# Autodesk Inventor assembly: Assembly2finalfinal
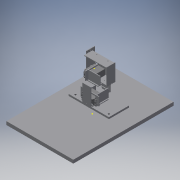
[picture p0: Inventor's stored thumbnail of the model, 180x180]
Saved by Autodesk Inventor 2019 (Build 230136000, 136)
## iProperties
Created: 2020-02-29
Part Number: Assembly2finalfinal
Document SubType Name: Assembly
Designer: Hp
Author: Hp
## Documents named in this file (14)
- C:\Users\Hp\Desktop\siri revant\final3ddiagrams\Assembly2finalfinal.iam
- C:\Users\Hp\Desktop\siri revant\final3ddiagrams\baseforclamp.ipt
- C:\Users\Hp\Desktop\siri revant\final3ddiagrams\basestand.ipt
- C:\Users\Hp\Desktop\siri revant\final3ddiagrams\clampforplatform.ipt
- C:\Users\Hp\Desktop\siri revant\final3ddiagrams\Lclamp1.ipt
- C:\Users\Hp\Desktop\siri revant\final3ddiagrams\Lclamp2.ipt
- C:\Users\Hp\Desktop\siri revant\final3ddiagrams\openslotforclamp.ipt
- C:\Users\Hp\Desktop\siri revant\final3ddiagrams\Part3.ipt
- C:\Users\Hp\Desktop\siri revant\final3ddiagrams\Part5.ipt
- C:\Users\Hp\Desktop\siri revant\final3ddiagrams\servostand.ipt
- C:\Users\Hp\Desktop\siri revant\final3ddiagrams\sidestandforservoclamp.ipt
- C:\Users\Hp\Downloads\HS-225MG.ipt
- C:\Users\Hp\Downloads\Ruderhorn.ipt
- C:\Users\Hp\Desktop\siri revant\final3ddiagrams\Part6.ipt
## Components (27 placed, 13 different names)
1. baseforclamp:1 — Rotational:2, Rigid:1, Rotational:7
2. basestand:1 — Rotational:1
3. clampforplatform:1 — Rotational:7, Rotational:8
4. Lclamp1:1 — Rotational:6, Rotational:9
5. openslotforclamp:1 — Rigid:1, Rotational:3, Rotational:4
6. Part3:1
7. Part5:1
8. servostand:1 — Rotational:1, Rotational:2, Rigid:2
9. sidestandforservoclamp:1 — Rotational:4
10. sidestandforservoclamp:2 — Rotational:3
11. HS-225MG:1 — Rigid:2, Rotational:5
12. Ruderhorn:1 — Rotational:5, Rotational:6
13. Lclamp1:2 — Rotational:8
14. Part6:1
15. Lclamp2:1 — Rotational:9, Rotational:10
16. baseforclamp:2 — Rotational:10, Rotational:11, Rotational:14, Rotational:16
17. clampforplatform:2 — Rotational:16, Rotational:18
18. Lclamp1:3 — Rotational:18, Rigid:3
19. Lclamp2:3 — Rigid:3
20. openslotforclamp:2 — Rotational:11, Rotational:12, Rotational:13
21. Part3:2
22. Part5:2
23. sidestandforservoclamp:3 — Rotational:12
24. sidestandforservoclamp:4 — Rotational:13
25. HS-225MG:2 — Rotational:14, Rotational:15
26. Ruderhorn:2 — Rotational:15, Rotational:17
27. Lclamp1:4 — Rotational:17
## Relationships (21: RevoluteJoint 18, WeldJoint 3)
- Rotational:1 [RevoluteJoint] (5 mm): basestand:1 ↔ servostand:1
- Rotational:2 [RevoluteJoint] (5 mm): baseforclamp:1 ↔ servostand:1
- Rigid:1 [WeldJoint]: baseforclamp:1 ↔ openslotforclamp:1
- Rotational:3 [RevoluteJoint]: openslotforclamp:1 ↔ sidestandforservoclamp:2
- Rotational:4 [RevoluteJoint]: openslotforclamp:1 ↔ sidestandforservoclamp:1
- Rigid:2 [WeldJoint] (5 mm): servostand:1 ↔ HS-225MG:1
- Rotational:5 [RevoluteJoint]: HS-225MG:1 ↔ Ruderhorn:1
- Rotational:6 [RevoluteJoint] (-2 mm): Lclamp1:1 ↔ Ruderhorn:1
- Rotational:7 [RevoluteJoint] (5 mm): baseforclamp:1 ↔ clampforplatform:1
- Rotational:8 [RevoluteJoint] (2 mm): clampforplatform:1 ↔ Lclamp1:2
- Rotational:9 [RevoluteJoint]: Lclamp1:1 ↔ Lclamp2:1
- Rotational:10 [RevoluteJoint] (2 mm): Lclamp2:1 ↔ baseforclamp:2
- Rotational:11 [RevoluteJoint]: baseforclamp:2 ↔ openslotforclamp:2
- Rotational:12 [RevoluteJoint]: openslotforclamp:2 ↔ sidestandforservoclamp:3
- Rotational:13 [RevoluteJoint]: openslotforclamp:2 ↔ sidestandforservoclamp:4
- Rotational:14 [RevoluteJoint]: baseforclamp:2 ↔ HS-225MG:2
- Rotational:15 [RevoluteJoint]: HS-225MG:2 ↔ Ruderhorn:2
- Rotational:16 [RevoluteJoint] (2 mm): baseforclamp:2 ↔ clampforplatform:2
- Rotational:17 [RevoluteJoint] (-3 mm): Ruderhorn:2 ↔ Lclamp1:4
- Rotational:18 [RevoluteJoint] (-2 mm): clampforplatform:2 ↔ Lclamp1:3
- Rigid:3 [WeldJoint]: Lclamp1:3 ↔ Lclamp2:3
